# Autodesk Inventor assembly: другая СОВЕРШЕННОЕ ТОЛСТАЯ
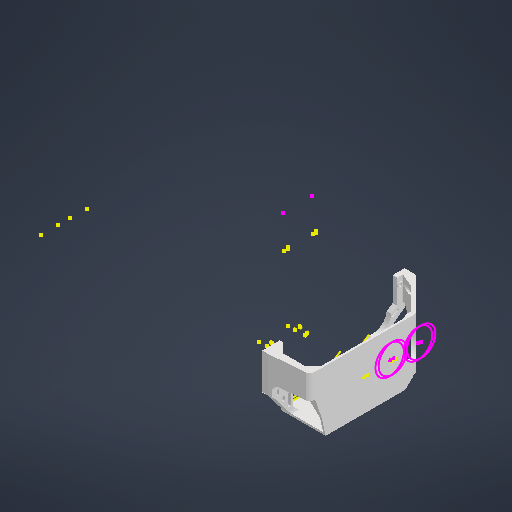
[picture p0: Inventor's stored thumbnail of the model, 512x512]
Saved by Autodesk Inventor 2025 (Build 290162000, 162)
## iProperties
Created: 2024-10-15
Part Number: другая СОВЕРШЕННОЕ ТОЛСТАЯ
Document SubType Name: Assembly
Designer: Phantom
Author: Phantom
## Documents named in this file (3)
- C:\Users\Phantom\Desktop\Phantom16950\другая СОВЕРШЕННОЕ ТОЛСТАЯ.iam
- C:\Users\Phantom\Desktop\Phantom16950\2 часть СОВЕРШЕННОЕ ТОЛСТАЯ .ipt
- C:\Users\Phantom\Desktop\Phantom16950\1 часть СОВЕРШЕННОЕ ТОЛСТАЯ .ipt
## Components (2 placed, 2 different names)
1. 2 часть СОВЕРШЕННОЕ ТОЛСТАЯ :1 — Совмещение:1, Заподлицо:1, Заподлицо:2
2. 1 часть СОВЕРШЕННОЕ ТОЛСТАЯ :1 — Совмещение:1, Заподлицо:1, Заподлицо:2
## Relationships (3: Flush 2, Mate 1)
- Совмещение:1 [Mate]: 2 часть СОВЕРШЕННОЕ ТОЛСТАЯ :1 ↔ 1 часть СОВЕРШЕННОЕ ТОЛСТАЯ :1
- Заподлицо:1 [Flush]: 2 часть СОВЕРШЕННОЕ ТОЛСТАЯ :1 ↔ 1 часть СОВЕРШЕННОЕ ТОЛСТАЯ :1
- Заподлицо:2 [Flush]: 2 часть СОВЕРШЕННОЕ ТОЛСТАЯ :1 ↔ 1 часть СОВЕРШЕННОЕ ТОЛСТАЯ :1
